# Autodesk Inventor assembly: noga_pre
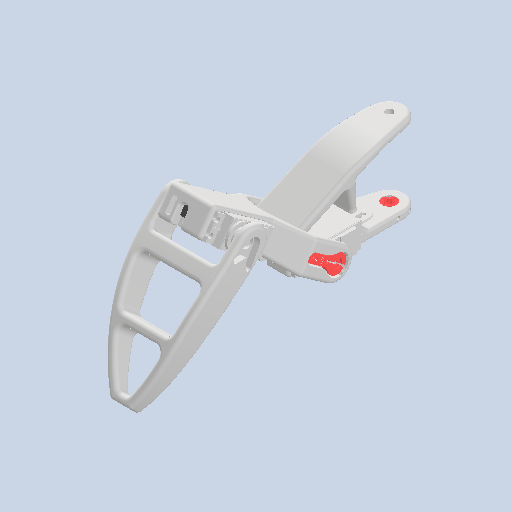
[picture p0: Inventor's stored thumbnail of the model, 512x512]
Saved by Autodesk Inventor 2023.4 (Build 274418000, 418)
## iProperties
Created: 2024-06-27
Part Number: noga_pre
Document SubType Name: Assembly
Designer: kamil
Author: kamil
## Documents named in this file (6)
- E:\PROJECTS_REPOS\Robal-2.0\mechanics\noga_pre.iam
- E:\PROJECTS_REPOS\Robal-2.0\mechanics\Standard-Servo.ipt
- E:\PROJECTS_REPOS\Robal-2.0\mechanics\czlon2_pre.ipt
- E:\PROJECTS_REPOS\Robal-2.0\mechanics\czlon3_pre.ipt
- E:\PROJECTS_REPOS\Robal-2.0\mechanics\czlon4_pre_2.ipt
- E:\PROJECTS_REPOS\Robal-2.0\mechanics\SERVO ARM HORN 25T ALUMINIUM\SERVO ARM HORN 25T ALUMINIUM.ipt
## Components (7 placed, 5 different names)
1. Standard-Servo:1 — Zestawiające:9, Zestawiające:10, Zestawiające:11, Mate:24, Mate:25, Mate:26
2. czlon2_pre:1 — Zestawiające:9, Zestawiające:10, Zestawiające:11, Angle:1, Mate:26, Mate:27, Mate:30
3. czlon3_pre:1 — Równoległe:4, Angle:2, Mate:27, Mate:28, Mate:29, Mate:30
4. Standard-Servo:3 — Równoległe:4, Zestawiające:22, Zestawiające:23, Mate:28, Mate:29
5. czlon4_pre_2:1 — Zestawiające:22, Zestawiające:23
6. SERVO ARM HORN 25T ALUMINIUM:1 — Angle:1
7. SERVO ARM HORN 25T ALUMINIUM:2 — Mate:24, Mate:25, Angle:2
## Relationships (15: Mate 12, Angle 2, Flush 1)
- Zestawiające:9 [Mate] (1 mm): Standard-Servo:1 ↔ czlon2_pre:1
- Zestawiające:10 [Mate] (1 mm): Standard-Servo:1 ↔ czlon2_pre:1
- Zestawiające:11 [Mate]: Standard-Servo:1 ↔ czlon2_pre:1
- Równoległe:4 [Flush]: czlon3_pre:1 ↔ Standard-Servo:3
- Zestawiające:22 [Mate] (2.1 mm): Standard-Servo:3 ↔ czlon4_pre_2:1
- Zestawiające:23 [Mate]: Standard-Servo:3 ↔ czlon4_pre_2:1
- Angle:1 (0 deg): czlon2_pre:1 ↔ SERVO ARM HORN 25T ALUMINIUM:1
- Mate:24: Standard-Servo:1 ↔ SERVO ARM HORN 25T ALUMINIUM:2
- Mate:25: Standard-Servo:1 ↔ SERVO ARM HORN 25T ALUMINIUM:2
- Mate:26: Standard-Servo:1 ↔ czlon2_pre:1
- Angle:2 (180 deg): czlon3_pre:1 ↔ SERVO ARM HORN 25T ALUMINIUM:2
- Mate:27: czlon2_pre:1 ↔ czlon3_pre:1
- Mate:28: czlon3_pre:1 ↔ Standard-Servo:3
- Mate:29: czlon3_pre:1 ↔ Standard-Servo:3
- Mate:30 (2 mm): czlon2_pre:1 ↔ czlon3_pre:1
